# Autodesk Inventor assembly: leg_Left_femur_ass
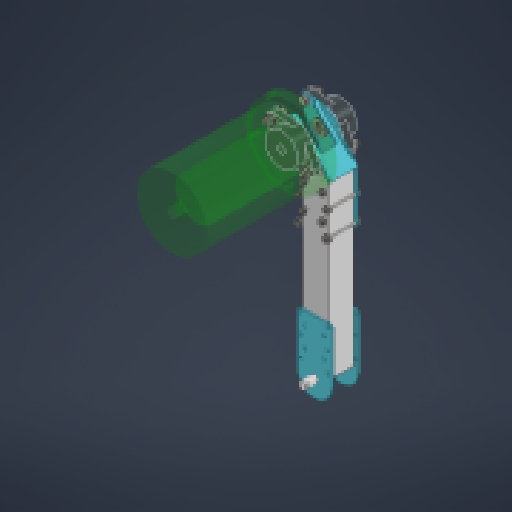
[picture p0: Inventor's stored thumbnail of the model, 512x512]
Saved by Autodesk Inventor 2026 (Build 300175000, 175)
## iProperties
Created: 2026-04-24
Part Number: leg_Left_femur_ass
Document SubType Name: Assembly
Designer: user
Mass: 1158.5 g
Surface Area: 2231.02 cm^2
Volume: 319.422 cm^3
Author: user
## Documents named in this file (14)
- C:\Users\user\vs_code_projects\ogonek-spider\physical-structure\cad\leg_femur\leg_Right_femur_ass.iam
- C:\Users\user\vs_code_projects\ogonek-spider\physical-structure\cad\leg_femur\femur_profile.ipt
- C:\Users\user\vs_code_projects\ogonek-spider\physical-structure\cad\leg_femur\femur_support_steel.ipt
- C:\Users\user\vs_code_projects\ogonek-spider\physical-structure\cad\leg_femur\femur_motor_steel.ipt
- C:\Users\user\vs_code_projects\ogonek-spider\physical-structure\cad\leg_femur\femur_outside_steel.ipt
- C:\Users\user\vs_code_projects\ogonek-spider\physical-structure\cad\leg_femur\shaft_femur.ipt
- C:\Users\user\vs_code_projects\ogonek-spider\physical-structure\cad\body_parts\motor_mass.ipt
- C:\Users\user\Documents\Inventor\Content Center Files\R2026\ru-RU\GOST 7872-89 (8000H)\Подшипник 8102H ГОСТ 7872-89.ipt
- C:\Users\user\vs_code_projects\ogonek-spider\physical-structure\cad\leg_femur\femur_reinforcement_tibea_steel.ipt
- C:\Users\user\vs_code_projects\ogonek-spider\physical-structure\cad\leg_femur\bearing_unit_15mm.ipt
- C:\Users\user\Documents\Inventor\Content Center Files\R2026\ru-RU\GOST 10338-80\Винт M10-6gx32 ГОСТ 10338-80.ipt
- C:\Users\user\Documents\Inventor\Content Center Files\R2026\ru-RU\Nut GOST R ISO 4161-2013\ГайкаM10-6H ГОСТ Р ISO 4161-2013.ipt
- C:\Users\user\Documents\Inventor\Content Center Files\R2026\ru-RU\Bolt 2 GOST 15591-70\Болт 2 M6×65 ГОСТ 15591-70.ipt
- C:\Users\user\Documents\Inventor\Content Center Files\R2026\ru-RU\Nut GOST R ISO 4161-2013\ГайкаM6-6H ГОСТ Р ISO 4161-2013.ipt
## Components (36 placed, 13 different names)
1. femur_profile:1 — Жесткий:2, Жесткий:3, С поворотом:1, С поворотом:2, С поворотом:3, С поворотом:4
2. femur_support_steel:1 — С поворотом:1, С поворотом:2, С поворотом:17, Жесткий:6, С поворотом:19, С поворотом:20, Совмещение:1, Совмещение:2, Совмещение:3, Совмещение:4, Совмещение:5, Совмещение:7, Совмещение:17, Совмещение:18, Совмещение:19, Совмещение:20, Совмещение:21, Совмещение:22, Совмещение:23, Совмещение:24, Совмещение:25, Совмещение:26, Совмещение:27, Совмещение:28, Совмещение:29, Совмещение:30, Совмещение:31, Совмещение:32, Совмещение:33, Совмещение:35, Совмещение:37, Совмещение:39, Совмещение:41, Совмещение:43, Совмещение:45, Совмещение:47
3. femur_motor_steel:1 — С поворотом:3, С поворотом:4, С поворотом:15, С поворотом:16, С поворотом:18, С поворотом:21, С поворотом:22, Совмещение:9, Совмещение:10, Совмещение:11, Совмещение:12, Совмещение:13, Совмещение:15, Совмещение:34, Совмещение:36, Совмещение:38, Совмещение:40, Совмещение:42, Совмещение:44, Совмещение:46, Совмещение:48
4. femur_outside_steel:1 — Жесткий:2
5. femur_outside_steel:2 — Жесткий:3, Жесткий:5
6. shaft_femur:1 — Жесткий:5
7. motor_mass:1 — С поворотом:15, С поворотом:16
8. Подшипник 8000H ГОСТ 7872-89 8102H:1 — С поворотом:17
9. Подшипник 8000H ГОСТ 7872-89 8102H:2 — С поворотом:18
10. femur_reinforcement_tibea_steel:1 — Жесткий:6
11. bearing_unit_15mm:1 — С поворотом:19, С поворотом:20, Совмещение:6, Совмещение:8
12. bearing_unit_15mm:2 — С поворотом:21, С поворотом:22, Совмещение:14, Совмещение:16
13. Винт ГОСТ 10338-80 M 10 x 32:1 — Совмещение:1, Совмещение:2
14. Гайка ГОСТ Р ISO 4161-2013 M10:1 — Совмещение:5, Совмещение:6
15. Винт ГОСТ 10338-80 M 10 x 32:2 — Совмещение:3, Совмещение:4
16. Гайка ГОСТ Р ISO 4161-2013 M10:2 — Совмещение:7, Совмещение:8
17. Винт ГОСТ 10338-80 M 10 x 32:3 — Совмещение:9, Совмещение:10
18. Гайка ГОСТ Р ISO 4161-2013 M10:3 — Совмещение:13, Совмещение:14
19. Винт ГОСТ 10338-80 M 10 x 32:4 — Совмещение:11, Совмещение:12
20. Гайка ГОСТ Р ISO 4161-2013 M10:4 — Совмещение:15, Совмещение:16
21. Болт 2 ГОСТ 15591-70 M6×65:1 — Совмещение:17, Совмещение:18
22. Гайка ГОСТ Р ISO 4161-2013 M6:1 — Совмещение:33, Совмещение:34
23. Болт 2 ГОСТ 15591-70 M6×65:2 — Совмещение:19, Совмещение:20
24. Болт 2 ГОСТ 15591-70 M6×65:3 — Совмещение:21, Совмещение:22
25. Болт 2 ГОСТ 15591-70 M6×65:4 — Совмещение:23, Совмещение:24
26. Болт 2 ГОСТ 15591-70 M6×65:5 — Совмещение:25, Совмещение:26
27. Болт 2 ГОСТ 15591-70 M6×65:6 — Совмещение:27, Совмещение:28
28. Болт 2 ГОСТ 15591-70 M6×65:7 — Совмещение:29, Совмещение:30
29. Болт 2 ГОСТ 15591-70 M6×65:8 — Совмещение:31, Совмещение:32
30. Гайка ГОСТ Р ISO 4161-2013 M6:2 — Совмещение:35, Совмещение:36
31. Гайка ГОСТ Р ISO 4161-2013 M6:3 — Совмещение:37, Совмещение:38
32. Гайка ГОСТ Р ISO 4161-2013 M6:4 — Совмещение:39, Совмещение:40
33. Гайка ГОСТ Р ISO 4161-2013 M6:5 — Совмещение:41, Совмещение:42
34. Гайка ГОСТ Р ISO 4161-2013 M6:6 — Совмещение:43, Совмещение:44
35. Гайка ГОСТ Р ISO 4161-2013 M6:7 — Совмещение:45, Совмещение:46
36. Гайка ГОСТ Р ISO 4161-2013 M6:8 — Совмещение:47, Совмещение:48
## Relationships (64: Mate 48, RevoluteJoint 12, WeldJoint 4)
- Жесткий:2 [WeldJoint]: femur_profile:1 ↔ femur_outside_steel:1
- Жесткий:3 [WeldJoint]: femur_profile:1 ↔ femur_outside_steel:2
- Жесткий:5 [WeldJoint] (20 mm): femur_outside_steel:2 ↔ shaft_femur:1
- С поворотом:1 [RevoluteJoint]: femur_profile:1 ↔ femur_support_steel:1
- С поворотом:2 [RevoluteJoint]: femur_profile:1 ↔ femur_support_steel:1
- С поворотом:3 [RevoluteJoint]: femur_profile:1 ↔ femur_motor_steel:1
- С поворотом:4 [RevoluteJoint]: femur_profile:1 ↔ femur_motor_steel:1
- С поворотом:15 [RevoluteJoint]: femur_motor_steel:1 ↔ motor_mass:1
- С поворотом:16 [RevoluteJoint]: femur_motor_steel:1 ↔ motor_mass:1
- С поворотом:17 [RevoluteJoint]: femur_support_steel:1 ↔ Подшипник 8000H ГОСТ 7872-89 8102H:1
- С поворотом:18 [RevoluteJoint]: femur_motor_steel:1 ↔ Подшипник 8000H ГОСТ 7872-89 8102H:2
- Жесткий:6 [WeldJoint]: femur_support_steel:1 ↔ femur_reinforcement_tibea_steel:1
- С поворотом:19 [RevoluteJoint]: femur_support_steel:1 ↔ bearing_unit_15mm:1
- С поворотом:20 [RevoluteJoint]: femur_support_steel:1 ↔ bearing_unit_15mm:1
- С поворотом:21 [RevoluteJoint]: femur_motor_steel:1 ↔ bearing_unit_15mm:2
- С поворотом:22 [RevoluteJoint]: femur_motor_steel:1 ↔ bearing_unit_15mm:2
- Совмещение:1 [Mate]: femur_support_steel:1 ↔ Винт ГОСТ 10338-80 M 10 x 32:1
- Совмещение:2 [Mate]: femur_support_steel:1 ↔ Винт ГОСТ 10338-80 M 10 x 32:1
- Совмещение:3 [Mate]: femur_support_steel:1 ↔ Винт ГОСТ 10338-80 M 10 x 32:2
- Совмещение:4 [Mate]: femur_support_steel:1 ↔ Винт ГОСТ 10338-80 M 10 x 32:2
- Совмещение:5 [Mate]: femur_support_steel:1 ↔ Гайка ГОСТ Р ISO 4161-2013 M10:1
- Совмещение:6 [Mate]: bearing_unit_15mm:1 ↔ Гайка ГОСТ Р ISO 4161-2013 M10:1
- Совмещение:7 [Mate]: femur_support_steel:1 ↔ Гайка ГОСТ Р ISO 4161-2013 M10:2
- Совмещение:8 [Mate]: bearing_unit_15mm:1 ↔ Гайка ГОСТ Р ISO 4161-2013 M10:2
- Совмещение:9 [Mate]: femur_motor_steel:1 ↔ Винт ГОСТ 10338-80 M 10 x 32:3
- Совмещение:10 [Mate]: femur_motor_steel:1 ↔ Винт ГОСТ 10338-80 M 10 x 32:3
- Совмещение:11 [Mate]: femur_motor_steel:1 ↔ Винт ГОСТ 10338-80 M 10 x 32:4
- Совмещение:12 [Mate]: femur_motor_steel:1 ↔ Винт ГОСТ 10338-80 M 10 x 32:4
- Совмещение:13 [Mate]: femur_motor_steel:1 ↔ Гайка ГОСТ Р ISO 4161-2013 M10:3
- Совмещение:14 [Mate]: bearing_unit_15mm:2 ↔ Гайка ГОСТ Р ISO 4161-2013 M10:3
- Совмещение:15 [Mate]: femur_motor_steel:1 ↔ Гайка ГОСТ Р ISO 4161-2013 M10:4
- Совмещение:16 [Mate]: bearing_unit_15mm:2 ↔ Гайка ГОСТ Р ISO 4161-2013 M10:4
- Совмещение:17 [Mate]: femur_support_steel:1 ↔ Болт 2 ГОСТ 15591-70 M6×65:1
- Совмещение:18 [Mate]: femur_support_steel:1 ↔ Болт 2 ГОСТ 15591-70 M6×65:1
- Совмещение:19 [Mate]: femur_support_steel:1 ↔ Болт 2 ГОСТ 15591-70 M6×65:2
- Совмещение:20 [Mate]: femur_support_steel:1 ↔ Болт 2 ГОСТ 15591-70 M6×65:2
- Совмещение:21 [Mate]: femur_support_steel:1 ↔ Болт 2 ГОСТ 15591-70 M6×65:3
- Совмещение:22 [Mate]: femur_support_steel:1 ↔ Болт 2 ГОСТ 15591-70 M6×65:3
- Совмещение:23 [Mate]: femur_support_steel:1 ↔ Болт 2 ГОСТ 15591-70 M6×65:4
- Совмещение:24 [Mate]: femur_support_steel:1 ↔ Болт 2 ГОСТ 15591-70 M6×65:4
- Совмещение:25 [Mate]: femur_support_steel:1 ↔ Болт 2 ГОСТ 15591-70 M6×65:5
- Совмещение:26 [Mate]: femur_support_steel:1 ↔ Болт 2 ГОСТ 15591-70 M6×65:5
- Совмещение:27 [Mate]: femur_support_steel:1 ↔ Болт 2 ГОСТ 15591-70 M6×65:6
- Совмещение:28 [Mate]: femur_support_steel:1 ↔ Болт 2 ГОСТ 15591-70 M6×65:6
- Совмещение:29 [Mate]: femur_support_steel:1 ↔ Болт 2 ГОСТ 15591-70 M6×65:7
- Совмещение:30 [Mate]: femur_support_steel:1 ↔ Болт 2 ГОСТ 15591-70 M6×65:7
- Совмещение:31 [Mate]: femur_support_steel:1 ↔ Болт 2 ГОСТ 15591-70 M6×65:8
- Совмещение:32 [Mate]: femur_support_steel:1 ↔ Болт 2 ГОСТ 15591-70 M6×65:8
- Совмещение:33 [Mate]: femur_support_steel:1 ↔ Гайка ГОСТ Р ISO 4161-2013 M6:1
- Совмещение:34 [Mate]: femur_motor_steel:1 ↔ Гайка ГОСТ Р ISO 4161-2013 M6:1
- Совмещение:35 [Mate]: femur_support_steel:1 ↔ Гайка ГОСТ Р ISO 4161-2013 M6:2
- Совмещение:36 [Mate]: femur_motor_steel:1 ↔ Гайка ГОСТ Р ISO 4161-2013 M6:2
- Совмещение:37 [Mate]: femur_support_steel:1 ↔ Гайка ГОСТ Р ISO 4161-2013 M6:3
- Совмещение:38 [Mate]: femur_motor_steel:1 ↔ Гайка ГОСТ Р ISO 4161-2013 M6:3
- Совмещение:39 [Mate]: femur_support_steel:1 ↔ Гайка ГОСТ Р ISO 4161-2013 M6:4
- Совмещение:40 [Mate]: femur_motor_steel:1 ↔ Гайка ГОСТ Р ISO 4161-2013 M6:4
- Совмещение:41 [Mate]: femur_support_steel:1 ↔ Гайка ГОСТ Р ISO 4161-2013 M6:5
- Совмещение:42 [Mate]: femur_motor_steel:1 ↔ Гайка ГОСТ Р ISO 4161-2013 M6:5
- Совмещение:43 [Mate]: femur_support_steel:1 ↔ Гайка ГОСТ Р ISO 4161-2013 M6:6
- Совмещение:44 [Mate]: femur_motor_steel:1 ↔ Гайка ГОСТ Р ISO 4161-2013 M6:6
- Совмещение:45 [Mate]: femur_support_steel:1 ↔ Гайка ГОСТ Р ISO 4161-2013 M6:7
- Совмещение:46 [Mate]: femur_motor_steel:1 ↔ Гайка ГОСТ Р ISO 4161-2013 M6:7
- Совмещение:47 [Mate]: femur_support_steel:1 ↔ Гайка ГОСТ Р ISO 4161-2013 M6:8
- Совмещение:48 [Mate]: femur_motor_steel:1 ↔ Гайка ГОСТ Р ISO 4161-2013 M6:8
